# Autodesk Inventor assembly: Assembly1
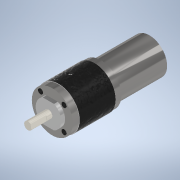
[picture p0: Inventor's stored thumbnail of the model, 180x180]
Saved by Autodesk Inventor 2020 (Build 240168000, 168)
## iProperties
Created: 2020-07-28
Part Number: Assembly1
Document SubType Name: Assembly
Designer: Ashiqrahman
Author: Ashiqrahman
## Documents named in this file (3)
- D:\projects\Intelligent Picking\my models\end effector motor\Assembly1.iam
- D:\projects\Intelligent Picking\my models\end effector motor\motor_body.ipt
- D:\projects\Intelligent Picking\my models\end effector motor\motor shaft.ipt
## Components (2 placed, 2 different names)
1. motor_body:1 — Flush:1
2. motor shaft:1 — Flush:1
## Relationships (1: Flush 1)
- Flush:1: motor_body:1 ↔ motor shaft:1
